# Autodesk Inventor assembly: Shaft Collar Metal
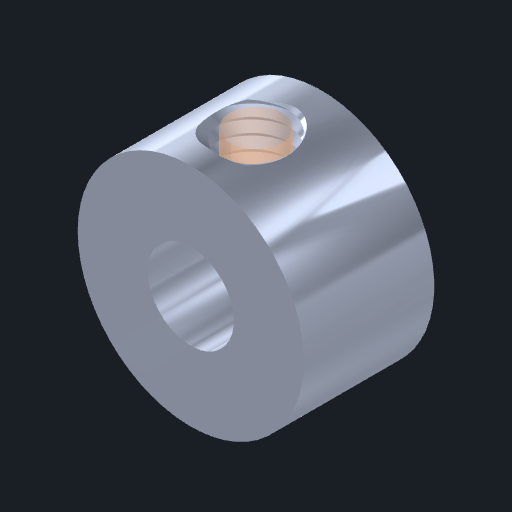
[picture p0: Inventor's stored thumbnail of the model, 512x512]
Saved by Autodesk Inventor 2023.2 (Build 272271000, 271)
## iProperties
Created: 2022-08-01
Part Number: Shaft Collar Metal
Document SubType Name: Assembly
Designer: ylu12
Author: ylu12
## Documents named in this file (15)
- D:\CAD\Parts\standard\Motion\Shafts\Shaft Collar.iam
- D:\CAD\Parts\standard\Motion\Shafts\Reference Parts\Shaft Collar Metal.ipt
- D:\CAD\Parts\standard\Motion\Shafts\Reference Parts\Set Screw.ipt
- D:\CAD\Parts\standard\Structure\Connectors\Screw Steel - Star\SScrew Hex Threaded .250.ipt
- D:\CAD\Parts\standard\Structure\Connectors\Screw Steel - Star\SScrew Star Threaded .250.ipt
- D:\CAD\Parts\standard\Structure\Connectors\Screw Steel - Star\SScrew Star Smooth .250.ipt
- D:\CAD\Parts\standard\Structure\Connectors\Screw Steel - Star\SScrew Hex Smooth .250.ipt
- D:\CAD\Parts\standard\Structure\Connectors\Screw Steel - Star.ipt
- D:\CAD\Parts\standard\Structure\Connectors\Screw Steel - Star\Screw Steel - Hex.ipt
- Shaft Collar Hex Smooth.iam
- Shaft Collar Hex Threaded.iam
- Shaft Collar No Screw.iam
- Shaft Collar Set Screw.iam
- Shaft Collar Star Smooth.iam
- Shaft Collar Star Threaded.iam
## Components (6 placed, 6 different names)
1. Shaft Collar Metal:1 — Mate:1, Mate:2, Flush:1, Insert:1, Insert:2, Insert:3, Insert:4, Insert:5
2. Set Screw:1 — Insert:1
3. SScrew Hex Threaded .250:1 — Insert:2
4. SScrew Star Threaded .250:1 — Insert:3
5. SScrew Hex Smooth .250:2 — Insert:5
6. SScrew Star Smooth .250:2 — Insert:4
## Relationships (8: Insert 5, Mate 2, Flush 1)
- Mate:1: Shaft Collar Metal:1
- Mate:2: Shaft Collar Metal:1
- Flush:1: Shaft Collar Metal:1
- Insert:1: Shaft Collar Metal:1 ↔ Set Screw:1
- Insert:2 (2.54 mm): Shaft Collar Metal:1 ↔ SScrew Hex Threaded .250:1
- Insert:3 (2.54 mm): Shaft Collar Metal:1 ↔ SScrew Star Threaded .250:1
- Insert:4 (2.54 mm): Shaft Collar Metal:1 ↔ SScrew Star Smooth .250:2
- Insert:5 (2.54 mm): Shaft Collar Metal:1 ↔ SScrew Hex Smooth .250:2
